# Autodesk Inventor assembly: Derive_BasePLate
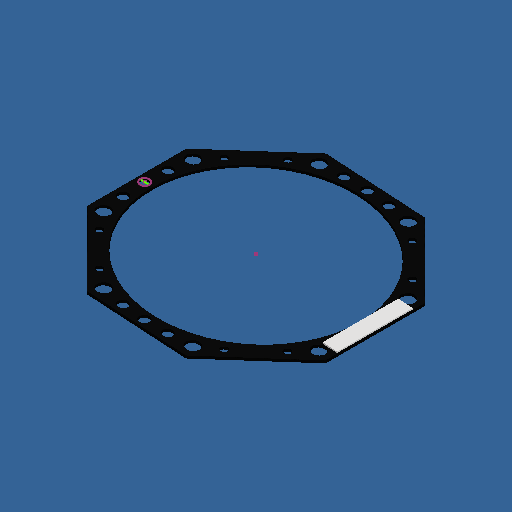
[picture p0: Inventor's stored thumbnail of the model, 512x512]
Saved by Autodesk Inventor 2026.2 (Build 302298000, 298)
## iProperties
Created: 2025-12-17
Part Number: Derive_BasePLate
Document SubType Name: Assembly
Designer: Thoma
Author: Thoma
## Documents named in this file (3)
- C:\Users\Thoma\OneDrive\Desktop\dir\telescope_cover\cover\Derive_Base_Plate.iam
- C:\Users\Thoma\OneDrive\Desktop\dir\telescope_cover\telescope\version_3\Telescope_End.ipt
- C:\Users\Thoma\OneDrive\Desktop\dir\telescope_cover\cover\Base_Plate_v1.ipt
## Components (2 placed, 2 different names)
1. Telescope_End:1 — Flush:1, Flush:2
2. Base_Plate_v1:1 — Flush:1, Flush:2
## Relationships (2: Flush 2)
- Flush:1: Telescope_End:1 ↔ Base_Plate_v1:1
- Flush:2 (1 mm): Telescope_End:1 ↔ Base_Plate_v1:1
